# Autodesk Inventor assembly: WCP Inline Elevator Bearing Block (WCP-0897)
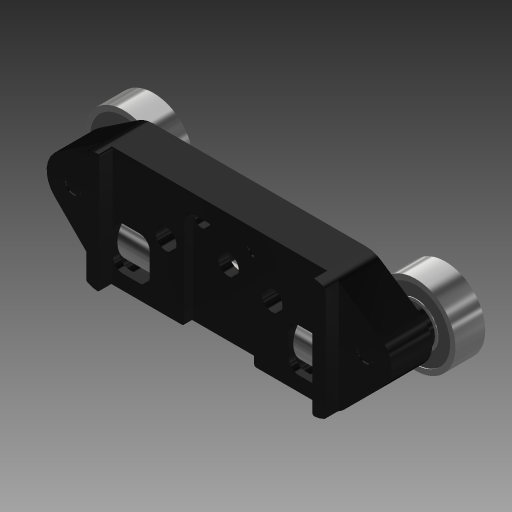
[picture p0: Inventor's stored thumbnail of the model, 512x512]
Saved by Autodesk Inventor 2023 (Build 270158000, 158)
## iProperties
Created: 2022-12-28
Part Number: WCP Inline Elevator Bearing Block (WCP-0897)
Document SubType Name: Assembly
Designer: Max Boord
Mass: 93.018 g
Surface Area: 152.431 cm^2
Volume: 19.9816 cm^3
Density: 4.65519 g/cm^3
Author: Max Boord
## Documents named in this file (9)
- E:\Collaborative Robots\Collaborative Part Library\Elevators\GreyT Elevator Parts\WCP Inline Elevator Bearing Block (WCP-0897).iam
- C:\Users\Max Boord\Desktop\WCP-0897\WCP-0897-001 Rev1.ipt
- E:\Collaborative Robots\Collaborative Part Library\Elevators\GreyT Elevator Parts\WCP-0039 Rev1.ipt
- C:\Users\Max Boord\Downloads\WCP-0473 Rev1.ipt
- E:\Collaborative Robots\Collaborative Part Library\Power Transfer\Bearings and Bushings\Bearings\R126.ipt
- E:\Collaborative Robots\Collaborative Part Library\Power Transfer\Bearings and Bushings\Bearings.ipt
- E:\Collaborative Robots\Collaborative Part Library\Power Transfer\Bearings and Bushings\Bearings\R4A.ipt
- E:\Collaborative Robots\Collaborative Part Library\Hardware\Dowel Pins\Dowel Pins.ipt
- E:\Collaborative Robots\Collaborative Part Library\Hardware\Dowel Pins\Dowel Pins\6mm x 2.25in Stainless Steel Dowel Pin.ipt
## Components (14 placed, 6 different names)
1. WCP-0897-001 Rev1:1 — Insert:1, Insert:2, Mate:1, Flush:1, Mate:2, Tangent:1, Mate:5, Mate:6
2. WCP-0039 Rev1:1 — Insert:7, Symmetry:1
3. WCP-0039 Rev1:2 — Insert:6
4. WCP-0473 Rev1:1 — Insert:2, Insert:3
5. WCP-0473 Rev1:2 — Insert:1, Insert:4
6. R126:1 — Insert:5, Insert:7, Mate:3, Symmetry:2
7. R126:2 — Insert:5, Insert:6, Symmetry:2
8. R4A:3 — Insert:4
9. R4A:4 — Insert:3
10. WCP-0039 Rev1:3
11. WCP-0039 Rev1:4 — Symmetry:1
12. R126:5 — Mate:4
13. R126:6
14. 6mm x 2.25in Stainless Steel Dowel Pin:1 — Mate:3, Mate:4, Tangent:1, Mate:5, Mate:6
## Relationships (20: Insert 10, Mate 6, Symmetry 2, Flush 1, Tangent 1)
- Insert:1: WCP-0897-001 Rev1:1 ↔ WCP-0473 Rev1:2
- Insert:2: WCP-0897-001 Rev1:1 ↔ WCP-0473 Rev1:1
- Insert:3: WCP-0473 Rev1:1 ↔ R4A:4
- Insert:4: WCP-0473 Rev1:2 ↔ R4A:3
- Insert:5: R126:1 ↔ R126:2
- Insert:6: WCP-0039 Rev1:2 ↔ R126:2
- Insert:7: WCP-0039 Rev1:1 ↔ R126:1
- [Insert]: R126:5 ↔ R126:6
- [Insert]: WCP-0039 Rev1:4 ↔ R126:6
- [Insert]: WCP-0039 Rev1:3 ↔ R126:5
- Mate:1: WCP-0897-001 Rev1:1
- Flush:1: WCP-0897-001 Rev1:1
- Mate:2: WCP-0897-001 Rev1:1
- Mate:3: R126:1 ↔ 6mm x 2.25in Stainless Steel Dowel Pin:1
- Mate:4: R126:5 ↔ 6mm x 2.25in Stainless Steel Dowel Pin:1
- Symmetry:1: WCP-0039 Rev1:1 ↔ WCP-0039 Rev1:4
- Tangent:1: WCP-0897-001 Rev1:1 ↔ 6mm x 2.25in Stainless Steel Dowel Pin:1
- Mate:5: WCP-0897-001 Rev1:1 ↔ 6mm x 2.25in Stainless Steel Dowel Pin:1
- Mate:6: WCP-0897-001 Rev1:1 ↔ 6mm x 2.25in Stainless Steel Dowel Pin:1
- Symmetry:2: R126:1 ↔ R126:2
## Named parameters: d7_d4 = 0 mm, d8_d5 = 0 mm, d9_d6 = 0 mm
